# Autodesk Inventor assembly: Tower Pro 9g Micro Servo SG90_MIR1
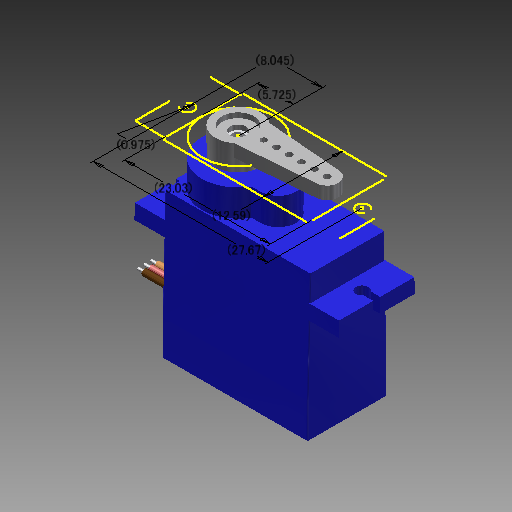
[picture p0: Inventor's stored thumbnail of the model, 512x512]
Saved by Autodesk Inventor 2017.3 (Build 213256000, 256)
## iProperties
Created: 2015-05-27
Part Number: Tower Pro 9g Micro Servo SG90_MIR1
Material: 一般
Document SubType Name: Assembly
Designer: sktom
Author: sktom
Sending System: SolidWorks 2014
Last Author: Simon
Last Saved: 2015-06-03
## Documents named in this file (3)
- D:\CloudStrage\OneDrive\CAD\MAJ\hackberry\HACKberry-hardware\3D_69%inlength\Inventor\HbHandForChild\servo\Tower Pro 9g Micro Servo SG90_MIR1.iam
- D:\CloudStrage\OneDrive\CAD\MAJ\hackberry\HACKberry-hardware\3D_69%inlength\Inventor\HbHandForChild\servo\Tower Pro 9g Micro Servo SG90_MIR1.ipt
- D:\CloudStrage\OneDrive\CAD\MAJ\hackberry\HACKberry-hardware\3D_69%inlength\Inventor\HbHandForChild\servo\SG90 plastic Horn_MIR1.ipt
## Components (2 placed, 2 different names)
1. Tower Pro 9g Micro Servo SG90_MIR1:1 — 挿入:1
2. SG90 plastic Horn_MIR1:1 — 挿入:1
## Relationships (1: Insert 1)
- 挿入:1 [Insert]: Tower Pro 9g Micro Servo SG90_MIR1:1 ↔ SG90 plastic Horn_MIR1:1
